# Autodesk Inventor assembly: Wentyl
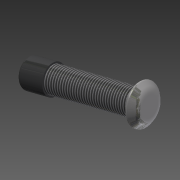
[picture p0: Inventor's stored thumbnail of the model, 180x180]
Saved by Autodesk Inventor 2015 (Build 190159000, 159)
## iProperties
Created: 2015-12-01
Part Number: Wentyl
Document SubType Name: Assembly
Designer: graaapsik
Author: graaapsik
## Documents named in this file (3)
- C:\Users\EriveltonDell\Documents\Centro Universitário da FEI\Wheelchair\CADEIRA DE RODAS - DESENHO\Model\Wentyl.iam
- C:\Users\EriveltonDell\Documents\Centro Universitário da FEI\Wheelchair\CADEIRA DE RODAS - DESENHO\Model\Rdzeń_wentyla.ipt
- C:\Users\EriveltonDell\Documents\Centro Universitário da FEI\Wheelchair\CADEIRA DE RODAS - DESENHO\Model\Nakrętka_wentyla.ipt
## Components (2 placed, 2 different names)
1. Rdzeń_wentyla:1 — Zestawiający:1, Zestawiający:2
2. Nakrętka_wentyla:1 — Zestawiający:1, Zestawiający:2
## Relationships (2: Mate 2)
- Zestawiający:1 [Mate]: Rdzeń_wentyla:1 ↔ Nakrętka_wentyla:1
- Zestawiający:2 [Mate]: Rdzeń_wentyla:1 ↔ Nakrętka_wentyla:1
